# Autodesk Inventor assembly: Ensamble final
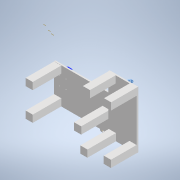
[picture p0: Inventor's stored thumbnail of the model, 180x180]
Saved by Autodesk Inventor 2020 (Build 240168000, 168)
## iProperties
Created: 2020-11-30
Part Number: Ensamble final
Document SubType Name: Assembly
Designer: Daniel
Author: Daniel
## Documents named in this file (9)
- D:\Desktop\Planos David Cifuentes\Ensamble final.iam
- D:\Desktop\Planos David Cifuentes\Estructura de soporte.ipt
- D:\Desktop\Planos David Cifuentes\Biela.ipt
- D:\Desktop\Planos David Cifuentes\Manivela.ipt
- D:\Desktop\Planos David Cifuentes\Punta de flecha.ipt
- D:\Desktop\Planos David Cifuentes\Eje principal.iam
- D:\Desktop\Planos David Cifuentes\Chumacera\SNLN 3024 + 23024 CCK_W33 + H 3024.ipt
- D:\Desktop\Planos David Cifuentes\Motor electrico - 1hp.ipt
- D:\Desktop\Planos David Cifuentes\Ensamble final\Design Accelerator\Banda V31.iam
## Components (8 placed, 8 different names)
1. Biela:1 — Rigid:1, Rotational:1
2. Manivela:1 — Rigid:1, Mate:7, Rigid:3
3. Punta de flecha:1 — Rotational:1
4. Eje principal:1 [sub-assembly] — Rigid:2, Mate:3, Mate:6, Mate:8, Rigid:3
5. SNLN 3024 + 23024 CCK_W33 + H 3024:1 — Mate:4, Mate:5, Mate:6, Mate:9, Mate:14
6. Motor electrico - 1hp:1 — Mate:1, Mate:2
7. Estructura de soporte:1 — Mate:1, Mate:2, Mate:5
8. Banda V3:1 [sub-assembly] — Rigid:2
## Relationships (14: Mate 10, WeldJoint 3, RevoluteJoint 1)
- Rigid:1 [WeldJoint]: Biela:1 ↔ Manivela:1
- Mate:1: Motor electrico - 1hp:1 ↔ Estructura de soporte:1
- Mate:2: Motor electrico - 1hp:1 ↔ Estructura de soporte:1
- Rigid:2 [WeldJoint]: Eje principal:1 ↔ Banda V3:1
- Mate:3: Eje principal:1
- Mate:4: SNLN 3024 + 23024 CCK_W33 + H 3024:1
- Mate:5: SNLN 3024 + 23024 CCK_W33 + H 3024:1 ↔ Estructura de soporte:1
- Mate:6: Eje principal:1 ↔ SNLN 3024 + 23024 CCK_W33 + H 3024:1
- Mate:7: Manivela:1
- Mate:8: Eje principal:1
- Rigid:3 [WeldJoint]: Manivela:1 ↔ Eje principal:1
- Mate:9: SNLN 3024 + 23024 CCK_W33 + H 3024:1
- Mate:14: SNLN 3024 + 23024 CCK_W33 + H 3024:1
- Rotational:1 [RevoluteJoint]: Biela:1 ↔ Punta de flecha:1
